# Autodesk Inventor assembly: Main_Assembly
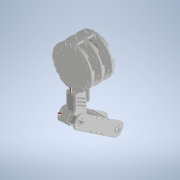
[picture p0: Inventor's stored thumbnail of the model, 180x180]
Saved by Autodesk Inventor 2020.1 (Build 241239000, 239)
## iProperties
Created: 2022-03-07
Part Number: Main_Assembly
Document SubType Name: Assembly
Designer: OEM
Author: OEM
## Documents named in this file (9)
- D:\Studia\Zebulon05\CAD\Main_Assembly.iam
- D:\Studia\Zebulon05\CAD\Body.ipt
- D:\Studia\Zebulon05\CAD\leg0.ipt
- D:\Studia\Zebulon05\CAD\Servo\HORN-D.ipt
- D:\Studia\Zebulon05\CAD\Servo\Case.ipt
- D:\Studia\Zebulon05\CAD\Leg1.ipt
- D:\Studia\Zebulon05\CAD\RPi Subs.ipt
- D:\Studia\Zebulon05\CAD\Spacer.ipt
- D:\Studia\Zebulon05\CAD\Leg2.ipt
## Components (18 placed, 10 different names)
1. Bod_lvl_plus1 — Mate:24, Mate:25, Mate:26, Mate:35, Mate:36, Mate:39
2. Body_lvl_Rpi — Mate:15, Mate:16, Mate:17, Mate:21, Mate:22, Mate:23, Mate:27, Mate:28, Mate:29, Mate:34, Mate:38, Mate:41, Mate:44, Mate:45, Mate:46, Mate:47
3. Body_lvl_FPGA — Mate:30, Mate:31, Mate:32, Mate:33, Mate:37, Mate:40, Mate:42, Mate:43
4. leg_part_0 — Mate:15, Mate:16, Mate:17, Mate:48, Mate:49, Mate:50
5. Leg_part_1 — Mate:51, Mate:52, Mate:53, Mate:54, Mate:55, Mate:56
6. Spacer:8 — Mate:33, Mate:34, Mate:37
7. Spacer:7 — Mate:39, Mate:41, Mate:44
8. Spacer:6 — Mate:35, Mate:36, Mate:38
9. Spacer:5 — Mate:40, Mate:42, Mate:43
10. Spacer:3 — Mate:21, Mate:22, Mate:23, Mate:24, Mate:25, Mate:26
11. Spacer:4 — Mate:27, Mate:28, Mate:29, Mate:30, Mate:31, Mate:32
12. RPi Subs:1 — Mate:45, Mate:46, Mate:47
13. Case:3 — Mate:8, Mate:9, Mate:51, Mate:52, Mate:53
14. HORN-D:1 — Mate:8, Mate:9, Mate:48, Mate:49, Mate:50
15. HORN-D:2 — Mate:13, Mate:14, Mate:58, Mate:59, Mate:60
16. Case:5 — Mate:13, Mate:14, Mate:54, Mate:55, Mate:56, Mate:57
17. Leg2:4 — Mate:61, Mate:62, Mate:63
18. Leg2:2 — Mate:57, Mate:58, Mate:59, Mate:60, Mate:61, Mate:62, Mate:63
## Relationships (50: Mate 50)
- Mate:8: Case:3 ↔ HORN-D:1
- Mate:9: Case:3 ↔ HORN-D:1
- Mate:13: HORN-D:2 ↔ Case:5
- Mate:14: HORN-D:2 ↔ Case:5
- Mate:15: Body_lvl_Rpi ↔ leg_part_0
- Mate:16: Body_lvl_Rpi ↔ leg_part_0
- Mate:17: Body_lvl_Rpi ↔ leg_part_0
- Mate:21: Body_lvl_Rpi ↔ Spacer:3
- Mate:22: Body_lvl_Rpi ↔ Spacer:3
- Mate:23: Body_lvl_Rpi ↔ Spacer:3
- Mate:24: Bod_lvl_plus1 ↔ Spacer:3
- Mate:25: Bod_lvl_plus1 ↔ Spacer:3
- Mate:26: Bod_lvl_plus1 ↔ Spacer:3
- Mate:27: Body_lvl_Rpi ↔ Spacer:4
- Mate:28: Body_lvl_Rpi ↔ Spacer:4
- Mate:29: Body_lvl_Rpi ↔ Spacer:4
- Mate:30: Body_lvl_FPGA ↔ Spacer:4
- Mate:31: Body_lvl_FPGA ↔ Spacer:4
- Mate:32: Body_lvl_FPGA ↔ Spacer:4
- Mate:33: Body_lvl_FPGA ↔ Spacer:8
- Mate:34: Body_lvl_Rpi ↔ Spacer:8
- Mate:35: Bod_lvl_plus1 ↔ Spacer:6
- Mate:36: Bod_lvl_plus1 ↔ Spacer:6
- Mate:37: Body_lvl_FPGA ↔ Spacer:8
- Mate:38: Body_lvl_Rpi ↔ Spacer:6
- Mate:39: Bod_lvl_plus1 ↔ Spacer:7
- Mate:40: Body_lvl_FPGA ↔ Spacer:5
- Mate:41: Body_lvl_Rpi ↔ Spacer:7
- Mate:42: Body_lvl_FPGA ↔ Spacer:5
- Mate:43: Body_lvl_FPGA ↔ Spacer:5
- Mate:44: Body_lvl_Rpi ↔ Spacer:7
- Mate:45: Body_lvl_Rpi ↔ RPi Subs:1
- Mate:46: Body_lvl_Rpi ↔ RPi Subs:1
- Mate:47: Body_lvl_Rpi ↔ RPi Subs:1
- Mate:48: leg_part_0 ↔ HORN-D:1
- Mate:49: leg_part_0 ↔ HORN-D:1
- Mate:50: leg_part_0 ↔ HORN-D:1
- Mate:51: Leg_part_1 ↔ Case:3
- Mate:52: Leg_part_1 ↔ Case:3
- Mate:53: Leg_part_1 ↔ Case:3
- Mate:54: Leg_part_1 ↔ Case:5
- Mate:55: Leg_part_1 ↔ Case:5
- Mate:56: Leg_part_1 ↔ Case:5
- Mate:57: Case:5 ↔ Leg2:2
- Mate:58: HORN-D:2 ↔ Leg2:2
- Mate:59: HORN-D:2 ↔ Leg2:2
- Mate:60: HORN-D:2 ↔ Leg2:2
- Mate:61: Leg2:4 ↔ Leg2:2
- Mate:62: Leg2:4 ↔ Leg2:2
- Mate:63: Leg2:4 ↔ Leg2:2
